# Autodesk Inventor assembly: 3136 1144 16-N
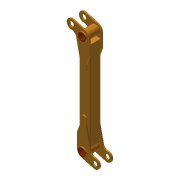
[picture p0: Inventor's stored thumbnail of the model, 180x180]
Saved by Autodesk Inventor 2022 Beta2 (Build 260130000, 130) ContinuousBuild 0
## iProperties
Shininess: 64.0
Length Units: 11269
Angle Units: 11279
Time Units: 11290
Mass Units: 11283
Length Display Precision: 3
Angle Display Precision: 2
Compacted: True
Created: 2003-04-13
Part Number: 3136 1144 16-N
Document SubType Name: Assembly
Designer: Uffe Bak
Density: 0.0
Volumn: 0.0
Area: 0.0
PropertySet Name: Model Information
Control State: 0
Master: False
Checked Out: False
Author: Uffe Bak
## Documents named in this file (4)
- C:\Autodesk Inventor 2021 Intro Practice Files\BOM\3136 1144 16-N.iam
- C:\Autodesk Inventor 2021 Intro Practice Files\BOM\3136 1133 80.iam
- C:\Autodesk Inventor 2021 Intro Practice Files\BOM\3136 1144 21.ipt
- C:\Autodesk Inventor 2021 Intro Practice Files\BOM\0500 4500 24.ipt
## Components (7 placed, 3 different names)
1. 3136 1133 80:1 [sub-assembly] — Insert:1, Insert:4
2. 3136 1144 21:1 — Insert:1, Insert:2, Insert:3
3. 3136 1144 21:2 — Insert:4, Insert:5, Insert:6
4. 0500 4500 24:1 — Insert:3
5. 0500 4500 24:2 — Insert:2
6. 0500 4500 24:3 — Insert:6
7. 0500 4500 24:4 — Insert:5
## Relationships (6: Insert 6)
- Insert:1: 3136 1133 80:1 ↔ 3136 1144 21:1
- Insert:2: 3136 1144 21:1 ↔ 0500 4500 24:2
- Insert:3: 3136 1144 21:1 ↔ 0500 4500 24:1
- Insert:4: 3136 1133 80:1 ↔ 3136 1144 21:2
- Insert:5: 3136 1144 21:2 ↔ 0500 4500 24:4
- Insert:6: 3136 1144 21:2 ↔ 0500 4500 24:3
